# Autodesk Inventor assembly: головаВерсия2
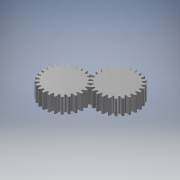
[picture p0: Inventor's stored thumbnail of the model, 180x180]
Saved by Autodesk Inventor 2019 (Build 230136000, 136)
## iProperties
Created: 2019-12-05
Part Number: головаВерсия2
Material: Типовые
Document SubType Name: Assembly
Designer: UlyaKZ
Author: UlyaKZ
## Documents named in this file (3)
- C:\Users\UlyaKZ\Desktop\RobotFix1\робот\головаВерсия2.iam
- C:\Users\UlyaKZ\Desktop\RobotFix1\робот\зубчатое колесо.ipt
- C:\Users\UlyaKZ\Desktop\RobotFix1\робот\головаВерсия2\Мастер проектирования\Цилиндрическое зубчатое зацепление1.iam
## Components (3 placed, 2 different names)
1. зубчатое колесо:1 — Заподлицо:1, Касательность:1, Совмещение:1, Совмещение:2
2. зубчатое колесо:2 — Заподлицо:1, Касательность:1, Совмещение:3, Совмещение:4
3. Цилиндрическое зубчатое зацепление:1 [sub-assembly] — Совмещение:1, Совмещение:2, Совмещение:3, Совмещение:4
## Relationships (6: Mate 4, Flush 1, Tangent 1)
- Заподлицо:1 [Flush]: зубчатое колесо:1 ↔ зубчатое колесо:2
- Касательность:1 [Tangent]: зубчатое колесо:1 ↔ зубчатое колесо:2
- Совмещение:1 [Mate]: зубчатое колесо:1 ↔ Цилиндрическое зубчатое зацепление:1
- Совмещение:2 [Mate]: зубчатое колесо:1 ↔ Цилиндрическое зубчатое зацепление:1
- Совмещение:3 [Mate]: зубчатое колесо:2 ↔ Цилиндрическое зубчатое зацепление:1
- Совмещение:4 [Mate]: зубчатое колесо:2 ↔ Цилиндрическое зубчатое зацепление:1
